# Autodesk Inventor assembly: simple_robot4
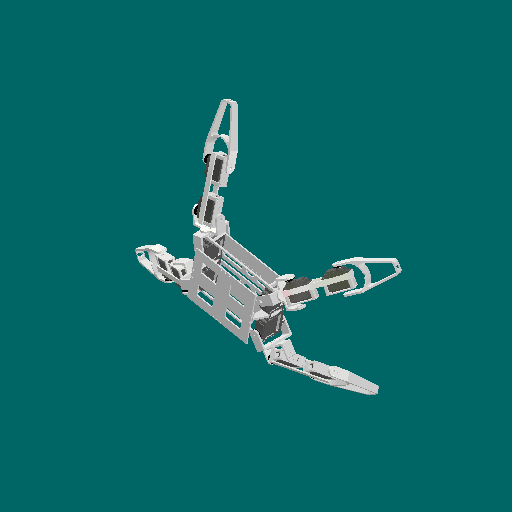
[picture p0: Inventor's stored thumbnail of the model, 512x512]
Saved by Autodesk Inventor 2026.1 (Build 301233000, 233)
## iProperties
Created: 2025-11-23
Part Number: simple_robot4
Document SubType Name: Assembly
Designer: emanuel
Author: emanuel
## Documents named in this file (5)
- C:\Users\emanuel\UnFolder\SpiderRobo\3dmodel\simple_robot4.iam
- C:\Users\emanuel\UnFolder\SpiderRobo\3dmodel\body4.ipt
- C:\Users\emanuel\UnFolder\SpiderRobo\3dmodel\coxa.ipt
- C:\Users\emanuel\UnFolder\SpiderRobo\3dmodel\femur4.ipt
- C:\Users\emanuel\UnFolder\SpiderRobo\3dmodel\smart_calf.ipt
## Components (13 placed, 4 different names)
1. body4:1 — Rotational:3, Rotational:6, Rotational:9, Rotational:12
2. coxa:1 — Rotational:11, Rotational:12
3. femur4:1 — Rotational:10, Rotational:11
4. smart_calf:1 — Rotational:10
5. coxa:2 — Rotational:8, Rotational:9
6. femur4:2 — Rotational:7, Rotational:8
7. smart_calf:2 — Rotational:7
8. coxa:3 — Rotational:2, Rotational:3
9. femur4:3 — Rotational:1, Rotational:2
10. smart_calf:3 — Rotational:1
11. coxa:4 — Rotational:5, Rotational:6
12. femur4:4 — Rotational:4, Rotational:5
13. smart_calf:4 — Rotational:4
## Relationships (12: RevoluteJoint 12)
- Rotational:1 [RevoluteJoint]: femur4:3 ↔ smart_calf:3
- Rotational:2 [RevoluteJoint]: coxa:3 ↔ femur4:3
- Rotational:3 [RevoluteJoint]: body4:1 ↔ coxa:3
- Rotational:4 [RevoluteJoint]: femur4:4 ↔ smart_calf:4
- Rotational:5 [RevoluteJoint]: coxa:4 ↔ femur4:4
- Rotational:6 [RevoluteJoint]: body4:1 ↔ coxa:4
- Rotational:7 [RevoluteJoint]: femur4:2 ↔ smart_calf:2
- Rotational:8 [RevoluteJoint]: coxa:2 ↔ femur4:2
- Rotational:9 [RevoluteJoint]: body4:1 ↔ coxa:2
- Rotational:10 [RevoluteJoint]: femur4:1 ↔ smart_calf:1
- Rotational:11 [RevoluteJoint]: coxa:1 ↔ femur4:1
- Rotational:12 [RevoluteJoint]: body4:1 ↔ coxa:1
